# Autodesk Inventor assembly: Pi_switch_assembly
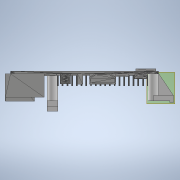
[picture p0: Inventor's stored thumbnail of the model, 180x180]
Saved by Autodesk Inventor 2022 (Build 260153000, 153)
## iProperties
Created: 2023-02-08
Part Number: Pi_switch_assembly
Document SubType Name: Assembly
Designer: scott
Author: scott
## Documents named in this file (4)
- C:\Users\scott\OneDrive\Documents\Cat project\Git_repository\Flinders_OpenCat\CAD components\Pi_switch_assembly.iam
- C:\Users\scott\OneDrive\Documents\Cat project\Git_repository\Flinders_OpenCat\CAD components\Imported Components\pi_v6\pi_v6.ipt
- C:\Users\scott\OneDrive\Documents\Cat project\Git_repository\Flinders_OpenCat\CAD components\Pi3B_spacer_F.ipt
- C:\Users\scott\OneDrive\Documents\Cat project\Git_repository\Flinders_OpenCat\CAD components\Pi3B_spacer_R.ipt
## Components (4 placed, 3 different names)
1. pi_v6:1 — Mate:1, Mate:2, Mate:3, Mate:4, Mate:5, Mate:6
2. Pi3B_spacer_F:1 — Mate:3, Mate:4, Flush:1, Angle:1
3. Pi3B_spacer_R:1 — Mate:1, Mate:2, Angle:1
4. Pi3B_spacer_F:2 — Mate:5, Mate:6, Flush:1
## Relationships (8: Mate 6, Flush 1, Angle 1)
- Mate:1: pi_v6:1 ↔ Pi3B_spacer_R:1
- Mate:2: pi_v6:1 ↔ Pi3B_spacer_R:1
- Mate:3: pi_v6:1 ↔ Pi3B_spacer_F:1
- Mate:4: pi_v6:1 ↔ Pi3B_spacer_F:1
- Mate:5: pi_v6:1 ↔ Pi3B_spacer_F:2
- Mate:6: pi_v6:1 ↔ Pi3B_spacer_F:2
- Flush:1: Pi3B_spacer_F:1 ↔ Pi3B_spacer_F:2
- Angle:1 (90 deg): Pi3B_spacer_F:1 ↔ Pi3B_spacer_R:1
